# Autodesk Inventor assembly: Stadio5
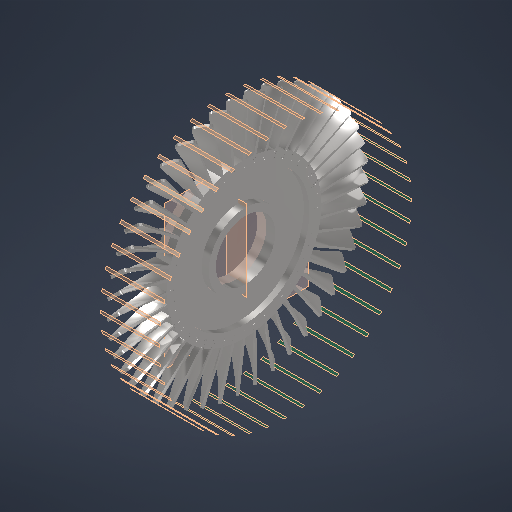
[picture p0: Inventor's stored thumbnail of the model, 512x512]
Saved by Autodesk Inventor 2026.2 (Build 302298010, 298A)
## iProperties
Created: 2026-04-23
Part Number: Stadio5
Document SubType Name: Assembly
Designer: Yan
Author: Yan
## Documents named in this file (3)
- C:\Users\Yan\Desktop\Turbina\Stadio5.iam
- C:\Users\Yan\Desktop\Turbina\DiscoPaleStadio5-DimensioniAprossimate.ipt
- C:\Users\Yan\Desktop\Turbina\PalaStadio5.ipt
## Components (45 placed, 2 different names)
1. DiscoPaleStadio5-DimensioniAprossimate:1 — Mate:1, Mate:2, Mate:3, Mate:4, Mate:5, Mate:6, Mate:7, Mate:8, Mate:9, Mate:10, Mate:11, Mate:12, Mate:13, Mate:14, Mate:15, Mate:16, Mate:17, Mate:18, Mate:19, Mate:20, Mate:21, Mate:22, Mate:23, Mate:24, Mate:25, Mate:26, Mate:27, Mate:28, Mate:29, Mate:30, Mate:31, Mate:32, Mate:33, Mate:34, Mate:35, Mate:36, Mate:37, Mate:38, Mate:39, Mate:40, Mate:41, Mate:42, Mate:43, Mate:44, Mate:45, Mate:46, Mate:47, Mate:48, Mate:49, Mate:50, Mate:51, Mate:52, Mate:53, Mate:54, Mate:55, Mate:56, Mate:57, Mate:58, Mate:59, Mate:60, Mate:61, Mate:62, Mate:63, Mate:64, Mate:65, Mate:66, Mate:67, Mate:68, Mate:69, Mate:70, Mate:71, Mate:72, Mate:73, Mate:74, Mate:75, Mate:76, Mate:77, Mate:78, Mate:79, Mate:80, Mate:81, Mate:82, Mate:83, Mate:84, Mate:85, Mate:86, Mate:87, Flush:1, Flush:2, Flush:3, Flush:4, Flush:5, Flush:6, Flush:7, Flush:8, Flush:9, Flush:10, Flush:11, Flush:12, Flush:13, Flush:14, Flush:15, Flush:16, Flush:17, Flush:18, Flush:19, Flush:20, Flush:21, Flush:22, Flush:23, Flush:24, Flush:25, Flush:26, Flush:27, Flush:28, Flush:29, Flush:30, Flush:31, Flush:32, Flush:33, Flush:34, Flush:35, Flush:36, Flush:37, Flush:38, Flush:39, Flush:40, Flush:41, Flush:42, Flush:43, Flush:44
2. PalaStadio5:1 — Mate:1, Mate:21, Flush:25
3. PalaStadio5:2 — Mate:2, Mate:22, Flush:24
4. PalaStadio5:3 — Mate:3, Mate:23, Flush:23
5. PalaStadio5:4 — Mate:4, Mate:24, Flush:22
6. PalaStadio5:5 — Mate:5, Mate:25, Flush:21
7. PalaStadio5:6 — Mate:6, Mate:26, Flush:20
8. PalaStadio5:7 — Mate:7, Mate:27, Flush:19
9. PalaStadio5:8 — Mate:8, Mate:28, Flush:18
10. PalaStadio5:9 — Mate:9, Mate:29, Flush:17
11. PalaStadio5:10 — Mate:10, Mate:30, Flush:16
12. PalaStadio5:11 — Mate:11, Mate:31, Flush:15
13. PalaStadio5:12 — Mate:12, Mate:32, Flush:14
14. PalaStadio5:13 — Mate:13, Mate:33, Flush:13
15. PalaStadio5:14 — Mate:14, Mate:34, Flush:12
16. PalaStadio5:15 — Mate:15, Mate:35, Flush:11
17. PalaStadio5:16 — Mate:16, Mate:36, Flush:10
18. PalaStadio5:17 — Mate:17, Mate:37, Flush:9
19. PalaStadio5:18 — Mate:18, Mate:38, Flush:8
20. PalaStadio5:19 — Mate:19, Mate:39, Flush:7
21. PalaStadio5:20 — Mate:20, Mate:40, Flush:6
22. PalaStadio5:21 — Mate:41, Mate:86, Flush:5
23. PalaStadio5:22 — Mate:42, Mate:87, Flush:4
24. PalaStadio5:23 — Mate:43, Mate:85, Flush:3
25. PalaStadio5:24 — Mate:44, Mate:84, Flush:2
26. PalaStadio5:25 — Mate:45, Mate:83, Flush:1
27. PalaStadio5:26 — Mate:46, Mate:82, Flush:44
28. PalaStadio5:27 — Mate:47, Mate:81, Flush:43
29. PalaStadio5:28 — Mate:48, Mate:80, Flush:42
30. PalaStadio5:29 — Mate:49, Mate:79, Flush:41
31. PalaStadio5:30 — Mate:50, Mate:78, Flush:40
32. PalaStadio5:31 — Mate:51, Flush:39
33. PalaStadio5:32 — Mate:52, Mate:77, Flush:38
34. PalaStadio5:33 — Mate:53, Mate:76, Flush:37
35. PalaStadio5:34 — Mate:54, Mate:75, Flush:36
36. PalaStadio5:35 — Mate:55, Mate:74, Flush:35
37. PalaStadio5:36 — Mate:56, Mate:73, Flush:34
38. PalaStadio5:37 — Mate:57, Mate:72, Flush:33
39. PalaStadio5:38 — Mate:58, Mate:71, Flush:32
40. PalaStadio5:39 — Mate:59, Mate:70, Flush:31
41. PalaStadio5:40 — Mate:60, Mate:69, Flush:30
42. PalaStadio5:41 — Mate:61, Mate:68, Flush:29
43. PalaStadio5:42 — Mate:62, Mate:67, Flush:28
44. PalaStadio5:43 — Mate:63, Mate:66, Flush:27
45. PalaStadio5:44 — Mate:64, Mate:65, Flush:26
## Relationships (131: Mate 87, Flush 44)
- Mate:1: DiscoPaleStadio5-DimensioniAprossimate:1 ↔ PalaStadio5:1
- Mate:2: DiscoPaleStadio5-DimensioniAprossimate:1 ↔ PalaStadio5:2
- Mate:3: DiscoPaleStadio5-DimensioniAprossimate:1 ↔ PalaStadio5:3
- Mate:4: DiscoPaleStadio5-DimensioniAprossimate:1 ↔ PalaStadio5:4
- Mate:5: DiscoPaleStadio5-DimensioniAprossimate:1 ↔ PalaStadio5:5
- Mate:6: DiscoPaleStadio5-DimensioniAprossimate:1 ↔ PalaStadio5:6
- Mate:7: DiscoPaleStadio5-DimensioniAprossimate:1 ↔ PalaStadio5:7
- Mate:8: DiscoPaleStadio5-DimensioniAprossimate:1 ↔ PalaStadio5:8
- Mate:9: DiscoPaleStadio5-DimensioniAprossimate:1 ↔ PalaStadio5:9
- Mate:10: DiscoPaleStadio5-DimensioniAprossimate:1 ↔ PalaStadio5:10
- Mate:11: DiscoPaleStadio5-DimensioniAprossimate:1 ↔ PalaStadio5:11
- Mate:12: DiscoPaleStadio5-DimensioniAprossimate:1 ↔ PalaStadio5:12
- Mate:13: DiscoPaleStadio5-DimensioniAprossimate:1 ↔ PalaStadio5:13
- Mate:14: DiscoPaleStadio5-DimensioniAprossimate:1 ↔ PalaStadio5:14
- Mate:15: DiscoPaleStadio5-DimensioniAprossimate:1 ↔ PalaStadio5:15
- Mate:16: DiscoPaleStadio5-DimensioniAprossimate:1 ↔ PalaStadio5:16
- Mate:17: DiscoPaleStadio5-DimensioniAprossimate:1 ↔ PalaStadio5:17
- Mate:18: DiscoPaleStadio5-DimensioniAprossimate:1 ↔ PalaStadio5:18
- Mate:19: DiscoPaleStadio5-DimensioniAprossimate:1 ↔ PalaStadio5:19
- Mate:20: DiscoPaleStadio5-DimensioniAprossimate:1 ↔ PalaStadio5:20
- Mate:21: DiscoPaleStadio5-DimensioniAprossimate:1 ↔ PalaStadio5:1
- Mate:22: DiscoPaleStadio5-DimensioniAprossimate:1 ↔ PalaStadio5:2
- Mate:23: DiscoPaleStadio5-DimensioniAprossimate:1 ↔ PalaStadio5:3
- Mate:24: DiscoPaleStadio5-DimensioniAprossimate:1 ↔ PalaStadio5:4
- Mate:25: DiscoPaleStadio5-DimensioniAprossimate:1 ↔ PalaStadio5:5
- Mate:26: DiscoPaleStadio5-DimensioniAprossimate:1 ↔ PalaStadio5:6
- Mate:27: DiscoPaleStadio5-DimensioniAprossimate:1 ↔ PalaStadio5:7
- Mate:28: DiscoPaleStadio5-DimensioniAprossimate:1 ↔ PalaStadio5:8
- Mate:29: DiscoPaleStadio5-DimensioniAprossimate:1 ↔ PalaStadio5:9
- Mate:30: DiscoPaleStadio5-DimensioniAprossimate:1 ↔ PalaStadio5:10
- Mate:31: DiscoPaleStadio5-DimensioniAprossimate:1 ↔ PalaStadio5:11
- Mate:32: DiscoPaleStadio5-DimensioniAprossimate:1 ↔ PalaStadio5:12
- Mate:33: DiscoPaleStadio5-DimensioniAprossimate:1 ↔ PalaStadio5:13
- Mate:34: DiscoPaleStadio5-DimensioniAprossimate:1 ↔ PalaStadio5:14
- Mate:35: DiscoPaleStadio5-DimensioniAprossimate:1 ↔ PalaStadio5:15
- Mate:36: DiscoPaleStadio5-DimensioniAprossimate:1 ↔ PalaStadio5:16
- Mate:37: DiscoPaleStadio5-DimensioniAprossimate:1 ↔ PalaStadio5:17
- Mate:38: DiscoPaleStadio5-DimensioniAprossimate:1 ↔ PalaStadio5:18
- Mate:39: DiscoPaleStadio5-DimensioniAprossimate:1 ↔ PalaStadio5:19
- Mate:40: DiscoPaleStadio5-DimensioniAprossimate:1 ↔ PalaStadio5:20
- Mate:41: DiscoPaleStadio5-DimensioniAprossimate:1 ↔ PalaStadio5:21
- Mate:42: DiscoPaleStadio5-DimensioniAprossimate:1 ↔ PalaStadio5:22
- Mate:43: DiscoPaleStadio5-DimensioniAprossimate:1 ↔ PalaStadio5:23
- Mate:44: DiscoPaleStadio5-DimensioniAprossimate:1 ↔ PalaStadio5:24
- Mate:45: DiscoPaleStadio5-DimensioniAprossimate:1 ↔ PalaStadio5:25
- Mate:46: DiscoPaleStadio5-DimensioniAprossimate:1 ↔ PalaStadio5:26
- Mate:47: DiscoPaleStadio5-DimensioniAprossimate:1 ↔ PalaStadio5:27
- Mate:48: DiscoPaleStadio5-DimensioniAprossimate:1 ↔ PalaStadio5:28
- Mate:49: DiscoPaleStadio5-DimensioniAprossimate:1 ↔ PalaStadio5:29
- Mate:50: DiscoPaleStadio5-DimensioniAprossimate:1 ↔ PalaStadio5:30
- Mate:51: DiscoPaleStadio5-DimensioniAprossimate:1 ↔ PalaStadio5:31
- Mate:52: DiscoPaleStadio5-DimensioniAprossimate:1 ↔ PalaStadio5:32
- Mate:53: DiscoPaleStadio5-DimensioniAprossimate:1 ↔ PalaStadio5:33
- Mate:54: DiscoPaleStadio5-DimensioniAprossimate:1 ↔ PalaStadio5:34
- Mate:55: DiscoPaleStadio5-DimensioniAprossimate:1 ↔ PalaStadio5:35
- Mate:56: DiscoPaleStadio5-DimensioniAprossimate:1 ↔ PalaStadio5:36
- Mate:57: DiscoPaleStadio5-DimensioniAprossimate:1 ↔ PalaStadio5:37
- Mate:58: DiscoPaleStadio5-DimensioniAprossimate:1 ↔ PalaStadio5:38
- Mate:59: DiscoPaleStadio5-DimensioniAprossimate:1 ↔ PalaStadio5:39
- Mate:60: DiscoPaleStadio5-DimensioniAprossimate:1 ↔ PalaStadio5:40
- Mate:61: DiscoPaleStadio5-DimensioniAprossimate:1 ↔ PalaStadio5:41
- Mate:62: DiscoPaleStadio5-DimensioniAprossimate:1 ↔ PalaStadio5:42
- Mate:63: DiscoPaleStadio5-DimensioniAprossimate:1 ↔ PalaStadio5:43
- Mate:64: DiscoPaleStadio5-DimensioniAprossimate:1 ↔ PalaStadio5:44
- Mate:65: DiscoPaleStadio5-DimensioniAprossimate:1 ↔ PalaStadio5:44
- Mate:66: DiscoPaleStadio5-DimensioniAprossimate:1 ↔ PalaStadio5:43
- Mate:67: DiscoPaleStadio5-DimensioniAprossimate:1 ↔ PalaStadio5:42
- Mate:68: DiscoPaleStadio5-DimensioniAprossimate:1 ↔ PalaStadio5:41
- Mate:69: DiscoPaleStadio5-DimensioniAprossimate:1 ↔ PalaStadio5:40
- Mate:70: DiscoPaleStadio5-DimensioniAprossimate:1 ↔ PalaStadio5:39
- Mate:71: DiscoPaleStadio5-DimensioniAprossimate:1 ↔ PalaStadio5:38
- Mate:72: DiscoPaleStadio5-DimensioniAprossimate:1 ↔ PalaStadio5:37
- Mate:73: DiscoPaleStadio5-DimensioniAprossimate:1 ↔ PalaStadio5:36
- Mate:74: DiscoPaleStadio5-DimensioniAprossimate:1 ↔ PalaStadio5:35
- Mate:75: DiscoPaleStadio5-DimensioniAprossimate:1 ↔ PalaStadio5:34
- Mate:76: DiscoPaleStadio5-DimensioniAprossimate:1 ↔ PalaStadio5:33
- Mate:77: DiscoPaleStadio5-DimensioniAprossimate:1 ↔ PalaStadio5:32
- Mate:78: DiscoPaleStadio5-DimensioniAprossimate:1 ↔ PalaStadio5:30
- Mate:79: DiscoPaleStadio5-DimensioniAprossimate:1 ↔ PalaStadio5:29
- Mate:80: DiscoPaleStadio5-DimensioniAprossimate:1 ↔ PalaStadio5:28
- Mate:81: DiscoPaleStadio5-DimensioniAprossimate:1 ↔ PalaStadio5:27
- Mate:82: DiscoPaleStadio5-DimensioniAprossimate:1 ↔ PalaStadio5:26
- Mate:83: DiscoPaleStadio5-DimensioniAprossimate:1 ↔ PalaStadio5:25
- Mate:84: DiscoPaleStadio5-DimensioniAprossimate:1 ↔ PalaStadio5:24
- Mate:85: DiscoPaleStadio5-DimensioniAprossimate:1 ↔ PalaStadio5:23
- Mate:86: DiscoPaleStadio5-DimensioniAprossimate:1 ↔ PalaStadio5:21
- Mate:87: DiscoPaleStadio5-DimensioniAprossimate:1 ↔ PalaStadio5:22
- Flush:1: DiscoPaleStadio5-DimensioniAprossimate:1 ↔ PalaStadio5:25
- Flush:2: DiscoPaleStadio5-DimensioniAprossimate:1 ↔ PalaStadio5:24
- Flush:3: DiscoPaleStadio5-DimensioniAprossimate:1 ↔ PalaStadio5:23
- Flush:4: DiscoPaleStadio5-DimensioniAprossimate:1 ↔ PalaStadio5:22
- Flush:5: DiscoPaleStadio5-DimensioniAprossimate:1 ↔ PalaStadio5:21
- Flush:6: DiscoPaleStadio5-DimensioniAprossimate:1 ↔ PalaStadio5:20
- Flush:7: DiscoPaleStadio5-DimensioniAprossimate:1 ↔ PalaStadio5:19
- Flush:8: DiscoPaleStadio5-DimensioniAprossimate:1 ↔ PalaStadio5:18
- Flush:9: DiscoPaleStadio5-DimensioniAprossimate:1 ↔ PalaStadio5:17
- Flush:10: DiscoPaleStadio5-DimensioniAprossimate:1 ↔ PalaStadio5:16
- Flush:11: DiscoPaleStadio5-DimensioniAprossimate:1 ↔ PalaStadio5:15
- Flush:12: DiscoPaleStadio5-DimensioniAprossimate:1 ↔ PalaStadio5:14
- Flush:13: DiscoPaleStadio5-DimensioniAprossimate:1 ↔ PalaStadio5:13
- Flush:14: DiscoPaleStadio5-DimensioniAprossimate:1 ↔ PalaStadio5:12
- Flush:15: DiscoPaleStadio5-DimensioniAprossimate:1 ↔ PalaStadio5:11
- Flush:16: DiscoPaleStadio5-DimensioniAprossimate:1 ↔ PalaStadio5:10
- Flush:17: DiscoPaleStadio5-DimensioniAprossimate:1 ↔ PalaStadio5:9
- Flush:18: DiscoPaleStadio5-DimensioniAprossimate:1 ↔ PalaStadio5:8
- Flush:19: DiscoPaleStadio5-DimensioniAprossimate:1 ↔ PalaStadio5:7
- Flush:20: DiscoPaleStadio5-DimensioniAprossimate:1 ↔ PalaStadio5:6
- Flush:21: DiscoPaleStadio5-DimensioniAprossimate:1 ↔ PalaStadio5:5
- Flush:22: DiscoPaleStadio5-DimensioniAprossimate:1 ↔ PalaStadio5:4
- Flush:23: DiscoPaleStadio5-DimensioniAprossimate:1 ↔ PalaStadio5:3
- Flush:24: DiscoPaleStadio5-DimensioniAprossimate:1 ↔ PalaStadio5:2
- Flush:25: DiscoPaleStadio5-DimensioniAprossimate:1 ↔ PalaStadio5:1
- Flush:26: DiscoPaleStadio5-DimensioniAprossimate:1 ↔ PalaStadio5:44
- Flush:27: DiscoPaleStadio5-DimensioniAprossimate:1 ↔ PalaStadio5:43
- Flush:28: DiscoPaleStadio5-DimensioniAprossimate:1 ↔ PalaStadio5:42
- Flush:29: DiscoPaleStadio5-DimensioniAprossimate:1 ↔ PalaStadio5:41
- Flush:30: DiscoPaleStadio5-DimensioniAprossimate:1 ↔ PalaStadio5:40
- Flush:31: DiscoPaleStadio5-DimensioniAprossimate:1 ↔ PalaStadio5:39
- Flush:32: DiscoPaleStadio5-DimensioniAprossimate:1 ↔ PalaStadio5:38
- Flush:33: DiscoPaleStadio5-DimensioniAprossimate:1 ↔ PalaStadio5:37
- Flush:34: DiscoPaleStadio5-DimensioniAprossimate:1 ↔ PalaStadio5:36
- Flush:35: DiscoPaleStadio5-DimensioniAprossimate:1 ↔ PalaStadio5:35
- Flush:36: DiscoPaleStadio5-DimensioniAprossimate:1 ↔ PalaStadio5:34
- Flush:37: DiscoPaleStadio5-DimensioniAprossimate:1 ↔ PalaStadio5:33
- Flush:38: DiscoPaleStadio5-DimensioniAprossimate:1 ↔ PalaStadio5:32
- Flush:39: DiscoPaleStadio5-DimensioniAprossimate:1 ↔ PalaStadio5:31
- Flush:40: DiscoPaleStadio5-DimensioniAprossimate:1 ↔ PalaStadio5:30
- Flush:41: DiscoPaleStadio5-DimensioniAprossimate:1 ↔ PalaStadio5:29
- Flush:42: DiscoPaleStadio5-DimensioniAprossimate:1 ↔ PalaStadio5:28
- Flush:43: DiscoPaleStadio5-DimensioniAprossimate:1 ↔ PalaStadio5:27
- Flush:44: DiscoPaleStadio5-DimensioniAprossimate:1 ↔ PalaStadio5:26
